# Autodesk Inventor assembly: BatteryCellAssembly
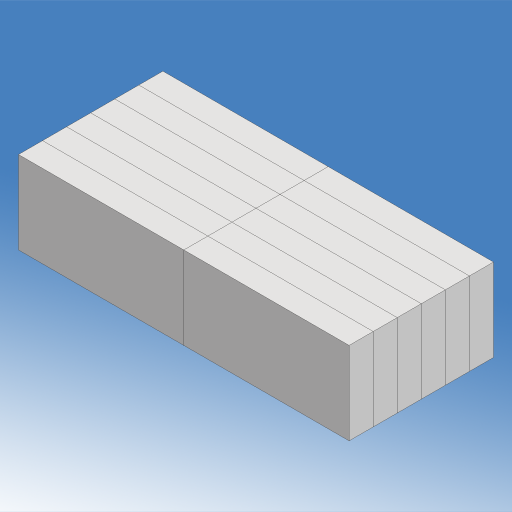
[picture p0: Inventor's stored thumbnail of the model, 512x512]
Saved by Autodesk Inventor 2024 (Build 280153000, 153)
## iProperties
Created: 2024-04-02
Part Number: BatteryCellAssembly
Document SubType Name: Assembly
Designer: seene
Author: seene
## Documents named in this file (2)
- C:\Users\seene\OneDrive\SBRT\Robocup Rescue\Chassis\Battery Drawer\BatteryCellAssembly.iam
- C:\Users\seene\OneDrive\SBRT\Robocup Rescue\Chassis\Electronics Box\EBox-Parts\Battery_Cell.ipt
## Components (12 placed, 1 different names)
1. Battery_Cell:1 — Flush:3, Mate:2, Mate:3, Flush:7, Flush:10
2. Battery_Cell:2 — Mate:10, Flush:11, Flush:20, Mate:11
3. Battery_Cell:3 — Flush:1, Mate:5, Flush:9, Flush:21, Flush:22
4. Battery_Cell:4 — Mate:9, Mate:10, Flush:11, Flush:12, Flush:19
5. Battery_Cell:5 — Mate:8, Mate:9, Flush:12, Flush:13, Flush:18, Flush:20
6. Battery_Cell:6 — Mate:7, Mate:8, Flush:13, Flush:14, Flush:17, Flush:19
7. Battery_Cell:7 — Mate:6, Mate:7, Flush:14, Flush:15, Flush:16
8. Battery_Cell:8 — Mate:6, Flush:15, Flush:16, Flush:17, Flush:18, Flush:21, Flush:22
9. Battery_Cell:9 — Flush:4, Mate:1, Mate:2, Flush:5, Flush:6
10. Battery_Cell:10 — Flush:2, Flush:3, Mate:3, Mate:4, Flush:6, Flush:7, Flush:8
11. Battery_Cell:11 — Flush:4, Mate:1, Flush:5, Flush:10, Mate:11
12. Battery_Cell:12 — Flush:1, Flush:2, Mate:4, Mate:5, Flush:8, Flush:9
## Relationships (33: Flush 22, Mate 11)
- Flush:1: Battery_Cell:3 ↔ Battery_Cell:12
- Flush:2: Battery_Cell:10 ↔ Battery_Cell:12
- Flush:3: Battery_Cell:1 ↔ Battery_Cell:10
- Flush:4: Battery_Cell:9 ↔ Battery_Cell:11
- Mate:1: Battery_Cell:9 ↔ Battery_Cell:11
- Mate:2: Battery_Cell:1 ↔ Battery_Cell:9
- Mate:3: Battery_Cell:1 ↔ Battery_Cell:10
- Mate:4: Battery_Cell:10 ↔ Battery_Cell:12
- Mate:5: Battery_Cell:3 ↔ Battery_Cell:12
- Flush:5: Battery_Cell:9 ↔ Battery_Cell:11
- Flush:6: Battery_Cell:9 ↔ Battery_Cell:10
- Flush:7: Battery_Cell:1 ↔ Battery_Cell:10
- Flush:8: Battery_Cell:10 ↔ Battery_Cell:12
- Flush:9: Battery_Cell:3 ↔ Battery_Cell:12
- Flush:10: Battery_Cell:1 ↔ Battery_Cell:11
- Mate:6: Battery_Cell:7 ↔ Battery_Cell:8
- Mate:7: Battery_Cell:6 ↔ Battery_Cell:7
- Mate:8: Battery_Cell:5 ↔ Battery_Cell:6
- Mate:9: Battery_Cell:4 ↔ Battery_Cell:5
- Mate:10: Battery_Cell:2 ↔ Battery_Cell:4
- Flush:11: Battery_Cell:2 ↔ Battery_Cell:4
- Flush:12: Battery_Cell:4 ↔ Battery_Cell:5
- Flush:13: Battery_Cell:5 ↔ Battery_Cell:6
- Flush:14: Battery_Cell:6 ↔ Battery_Cell:7
- Flush:15: Battery_Cell:7 ↔ Battery_Cell:8
- Flush:16: Battery_Cell:7 ↔ Battery_Cell:8
- Flush:17: Battery_Cell:6 ↔ Battery_Cell:8
- Flush:18: Battery_Cell:5 ↔ Battery_Cell:8
- Flush:19: Battery_Cell:4 ↔ Battery_Cell:6
- Flush:20: Battery_Cell:2 ↔ Battery_Cell:5
- Mate:11: Battery_Cell:2 ↔ Battery_Cell:11
- Flush:21: Battery_Cell:3 ↔ Battery_Cell:8
- Flush:22: Battery_Cell:3 ↔ Battery_Cell:8
